# Autodesk Inventor assembly: Shifter
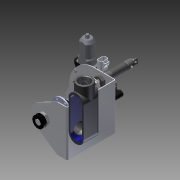
[picture p0: Inventor's stored thumbnail of the model, 180x180]
Saved by Autodesk Inventor 2015 (Build 190159000, 159)
## iProperties
Created: 2015-01-23
Part Number: Shifter
Document SubType Name: Assembly
Designer: Guest
Author: Guest
## Documents named in this file (22)
- C:\Users\Brian\Documents\GitHub\FIRST-Team-1719-CAD-Team\2015 Robot CAD\Devices\Extender\Shifter\Shifter.iam
- C:\Users\Brian\Documents\GitHub\FIRST-Team-1719-CAD-Team\2015 Robot CAD\Devices\Extender\Shifter\ND Motor Left.ipt
- C:\Users\Brian\Documents\GitHub\FIRST-Team-1719-CAD-Team\2015 Robot CAD\Devices\Extender\Shifter\Motor Mount.ipt
- C:\Users\Brian\Documents\GitHub\FIRST-Team-1719-CAD-Team\2015 Robot CAD\Devices\Extender\Shifter\Motor Bolt Nut.ipt
- C:\Users\Brian\Documents\GitHub\FIRST-Team-1719-CAD-Team\2015 Robot CAD\Devices\Extender\Shifter\Motor Bolt.ipt
- C:\Users\Brian\Documents\GitHub\FIRST-Team-1719-CAD-Team\2015 Robot CAD\Devices\Extender\Shifter\Piston\D_9.ipt
- C:\Users\Brian\Documents\GitHub\FIRST-Team-1719-CAD-Team\2015 Robot CAD\Devices\Extender\Shifter\Piston.iam
- C:\Users\Brian\Documents\GitHub\FIRST-Team-1719-CAD-Team\2015 Robot CAD\Devices\Extender\Shifter\Hub.ipt
- C:\Users\Brian\Documents\GitHub\FIRST-Team-1719-CAD-Team\2015 Robot CAD\Devices\Extender\Shifter\Access Fitting.ipt
- C:\Users\Brian\Documents\GitHub\FIRST-Team-1719-CAD-Team\2015 Robot CAD\Devices\Extender\Shifter\Piston Bore Nut.ipt
- C:\Users\Brian\Documents\GitHub\FIRST-Team-1719-CAD-Team\2015 Robot CAD\Devices\Extender\Shifter\Bottom Hub Plate.ipt
- C:\Users\Brian\Documents\GitHub\FIRST-Team-1719-CAD-Team\2015 Robot CAD\Devices\Extender\Shifter\Spacer.ipt
- C:\Users\Brian\Documents\GitHub\FIRST-Team-1719-CAD-Team\2015 Robot CAD\Devices\Extender\Shifter\Upper Hub Plate.ipt
- C:\Users\Brian\Documents\GitHub\FIRST-Team-1719-CAD-Team\2015 Robot CAD\Devices\Extender\Shifter\Flanged Bushing.ipt
- C:\Users\Brian\Documents\GitHub\FIRST-Team-1719-CAD-Team\2015 Robot CAD\Devices\Extender\Shifter\1 4-20 Bolt.ipt
- C:\Users\Brian\Documents\GitHub\FIRST-Team-1719-CAD-Team\2015 Robot CAD\Devices\Extender\Shifter\1 4-20 Nut.ipt
- C:\Users\Brian\Documents\GitHub\FIRST-Team-1719-CAD-Team\2015 Robot CAD\Devices\Extender\Shifter\625 Key Hub.ipt
- C:\Users\Brian\Documents\GitHub\FIRST-Team-1719-CAD-Team\2015 Robot CAD\Devices\Extender\Shifter\5 16 Shaft.ipt
- C:\Users\Brian\Documents\GitHub\FIRST-Team-1719-CAD-Team\2015 Robot CAD\Devices\Extender\Shifter\Shaft Collar.ipt
- C:\Users\Brian\Documents\GitHub\FIRST-Team-1719-CAD-Team\2015 Robot CAD\Devices\Extender\Shifter\Bearing.ipt
- C:\Users\Brian\Documents\GitHub\FIRST-Team-1719-CAD-Team\2015 Robot CAD\Devices\Extender\Shifter\Hub Key.ipt
- C:\Users\Brian\Documents\GitHub\FIRST-Team-1719-CAD-Team\2015 Robot CAD\Devices\Extender\Shifter\Spool Key.ipt
## Components (38 placed, 21 different names)
1. ND Motor Left:1 — Flush:1, Mate:5, Mate:8, Mate:9, Mate:17, Mate:63, Mate:68
2. Motor Mount:1 — Flush:1, Mate:1, Mate:2, Mate:3, Mate:4, Mate:13, Mate:14, Mate:15, Mate:16, Mate:55, Angle:4, Mate:62, Angle:8, Angle:9
3. Motor Bolt Nut:1 — Mate:5, Mate:6
4. Motor Bolt Nut:2 — Mate:7, Mate:8
5. Motor Bolt:1 — Flush:2, Mate:1, Mate:2, Mate:10, Mate:68
6. Motor Bolt:2 — Flush:3, Mate:4, Mate:6
7. Motor Bolt:3 — Flush:2, Flush:3, Mate:3, Mate:7, Mate:63
8. Motor Bolt Nut:3 — Mate:9, Mate:10
9. D_9:1 — Mate:11, Flush:5, Mate:16
10. Piston:1 [sub-assembly] — Flush:4, Mate:11, Mate:13, Mate:14, Angle:1, Mate:20, Mate:24, Flush:9, Angle:5, Mate:67, Flush:17, Mate:69
11. D_9:2 — Mate:12, Flush:5
12. Piston:2 [sub-assembly] — Flush:4, Mate:12, Mate:15, Angle:1, Mate:18, Mate:22, Flush:17
13. Hub:1 — Mate:17, Mate:31, Mate:42, Angle:2, Mate:52, Angle:3
14. Piston Bore Nut:1 — Mate:18
15. Piston Bore Nut:2 — Mate:20, Flush:6, Mate:69
16. Piston Bore Nut:3 — Mate:22, Mate:23
17. Piston Bore Nut:4 — Mate:24, Mate:25, Flush:9
18. Bottom Hub Plate:1 — Flush:6, Mate:23, Mate:25, Flush:7, Mate:36, Mate:64, Mate:65, Mate:67
19. Spacer:1 — Flush:7, Flush:8, Mate:27, Mate:28, Mate:64, Mate:65
20. Upper Hub Plate:1 — Flush:8, Mate:27, Mate:28, Mate:29, Mate:30, Mate:31, Mate:32, Mate:33, Mate:34, Mate:35, Mate:39
21. Flanged Bushing:1 — Mate:29, Mate:30, Mate:54, Mate:66
22. 1 4-20 Bolt:1 — Flush:12, Mate:34, Mate:38
23. 1 4-20 Bolt:2 — Flush:10, Mate:33, Mate:41
24. 1 4-20 Bolt:3 — Flush:11, Flush:12, Mate:35, Mate:37
25. 1 4-20 Bolt:4 — Flush:10, Flush:11, Mate:32, Mate:36, Mate:40
26. 1 4-20 Nut:1 — Flush:13, Flush:14, Mate:39, Mate:40
27. 1 4-20 Nut:2 — Flush:14, Flush:15, Mate:38
28. 1 4-20 Nut:3 — Flush:15, Mate:37
29. 1 4-20 Nut:4 — Flush:13, Mate:41
30. 625 Key Hub:1 — Mate:42, Mate:43, Mate:44, Flush:16, Mate:45, Mate:46, Mate:56
31. 625 Key Hub:2 — Mate:43, Mate:44, Flush:16, Angle:2, Mate:48, Mate:49, Mate:50
32. 5 16 Shaft:1 — Mate:52, Angle:3, Mate:57, Angle:6, Angle:7, Mate:66, Flush:19, Angle:9, Mate:70, Mate:71
33. Shaft Collar:1 — Mate:45, Mate:46, Mate:54, Angle:7, Mate:73
34. Shaft Collar:2 — Mate:48, Mate:51, Angle:6, Flush:19, Mate:58
35. Bearing:1 — Mate:49, Mate:50, Mate:51, Mate:62, Mate:72
36. Access Fitting:1 — Mate:55, Mate:56, Mate:61, Angle:8
37. Hub Key:1 — Flush:20, Flush:21, Mate:71, Mate:73
38. Spool Key:1 — Flush:20, Flush:21, Mate:70, Mate:72
## Relationships (97: Mate 68, Flush 20, Angle 9)
- Flush:1: ND Motor Left:1 ↔ Motor Mount:1
- Flush:2: Motor Bolt:1 ↔ Motor Bolt:3
- Flush:3: Motor Bolt:2 ↔ Motor Bolt:3
- Mate:1: Motor Mount:1 ↔ Motor Bolt:1
- Mate:2: Motor Mount:1 ↔ Motor Bolt:1
- Mate:3: Motor Mount:1 ↔ Motor Bolt:3
- Mate:4: Motor Mount:1 ↔ Motor Bolt:2
- Mate:5: ND Motor Left:1 ↔ Motor Bolt Nut:1
- Mate:6: Motor Bolt Nut:1 ↔ Motor Bolt:2
- Mate:7: Motor Bolt Nut:2 ↔ Motor Bolt:3
- Mate:8: ND Motor Left:1 ↔ Motor Bolt Nut:2
- Mate:9: ND Motor Left:1 ↔ Motor Bolt Nut:3
- Mate:10: Motor Bolt:1 ↔ Motor Bolt Nut:3
- Flush:4: Piston:1 ↔ Piston:2
- Mate:11: D_9:1 ↔ Piston:1
- Mate:12: D_9:2 ↔ Piston:2
- Mate:13: Motor Mount:1 ↔ Piston:1
- Mate:14: Motor Mount:1 ↔ Piston:1
- Mate:15: Motor Mount:1 ↔ Piston:2
- Flush:5: D_9:1 ↔ D_9:2
- Mate:16: Motor Mount:1 ↔ D_9:1
- Angle:1 (0 deg): Piston:1 ↔ Piston:2
- Mate:17: ND Motor Left:1 ↔ Hub:1
- Mate:18: Piston:2 ↔ Piston Bore Nut:1
- Mate:20: Piston:1 ↔ Piston Bore Nut:2
- Flush:6: Piston Bore Nut:2 ↔ Bottom Hub Plate:1
- Mate:22: Piston:2 ↔ Piston Bore Nut:3
- Mate:23: Piston Bore Nut:3 ↔ Bottom Hub Plate:1
- Mate:24: Piston:1 ↔ Piston Bore Nut:4
- Mate:25: Piston Bore Nut:4 ↔ Bottom Hub Plate:1
- Flush:7: Bottom Hub Plate:1 ↔ Spacer:1
- Flush:8: Spacer:1 ↔ Upper Hub Plate:1
- Mate:27: Spacer:1 ↔ Upper Hub Plate:1
- Mate:28: Spacer:1 ↔ Upper Hub Plate:1
- Flush:9 (-2.4892 mm): Piston:1 ↔ Piston Bore Nut:4
- Mate:29: Upper Hub Plate:1 ↔ Flanged Bushing:1
- Mate:30: Upper Hub Plate:1 ↔ Flanged Bushing:1
- Mate:31 (6.35 mm): Hub:1 ↔ Upper Hub Plate:1
- Flush:10: 1 4-20 Bolt:2 ↔ 1 4-20 Bolt:4
- Flush:11: 1 4-20 Bolt:3 ↔ 1 4-20 Bolt:4
- Flush:12: 1 4-20 Bolt:1 ↔ 1 4-20 Bolt:3
- Mate:32: Upper Hub Plate:1 ↔ 1 4-20 Bolt:4
- Mate:33: Upper Hub Plate:1 ↔ 1 4-20 Bolt:2
- Mate:34: Upper Hub Plate:1 ↔ 1 4-20 Bolt:1
- Mate:35: Upper Hub Plate:1 ↔ 1 4-20 Bolt:3
- Mate:36: Bottom Hub Plate:1 ↔ 1 4-20 Bolt:4
- Flush:13: 1 4-20 Nut:1 ↔ 1 4-20 Nut:4
- Flush:14: 1 4-20 Nut:1 ↔ 1 4-20 Nut:2
- Flush:15: 1 4-20 Nut:2 ↔ 1 4-20 Nut:3
- Mate:37: 1 4-20 Bolt:3 ↔ 1 4-20 Nut:3
- Mate:38: 1 4-20 Bolt:1 ↔ 1 4-20 Nut:2
- Mate:39: Upper Hub Plate:1 ↔ 1 4-20 Nut:1
- Mate:40: 1 4-20 Bolt:4 ↔ 1 4-20 Nut:1
- Mate:41: 1 4-20 Bolt:2 ↔ 1 4-20 Nut:4
- Mate:42: Hub:1 ↔ 625 Key Hub:1
- Mate:43: 625 Key Hub:1 ↔ 625 Key Hub:2
- Mate:44: 625 Key Hub:1 ↔ 625 Key Hub:2
- Flush:16: 625 Key Hub:1 ↔ 625 Key Hub:2
- Angle:2 (0 deg): Hub:1 ↔ 625 Key Hub:2
- Mate:45: 625 Key Hub:1 ↔ Shaft Collar:1
- Mate:46: 625 Key Hub:1 ↔ Shaft Collar:1
- Mate:48: 625 Key Hub:2 ↔ Shaft Collar:2
- Mate:49: 625 Key Hub:2 ↔ Bearing:1
- Mate:50: 625 Key Hub:2 ↔ Bearing:1
- Mate:51: Shaft Collar:2 ↔ Bearing:1
- Mate:52: Hub:1 ↔ 5 16 Shaft:1
- Angle:3 (0 deg): Hub:1 ↔ 5 16 Shaft:1
- Mate:54 (25.4 mm): Flanged Bushing:1 ↔ Shaft Collar:1
- Mate:55: Motor Mount:1 ↔ Access Fitting:1
- Mate:56 (-25.4 mm): 625 Key Hub:1 ↔ Access Fitting:1
- Mate:57: 5 16 Shaft:1
- Mate:58: Shaft Collar:2
- Mate:59
- Mate:60
- Angle:4 (0 deg): Motor Mount:1
- Mate:61: Access Fitting:1
- Mate:62: Motor Mount:1 ↔ Bearing:1
- Mate:63: ND Motor Left:1 ↔ Motor Bolt:3
- Angle:5 (0 deg): Piston:1
- Angle:6 (0 deg): 5 16 Shaft:1 ↔ Shaft Collar:2
- Angle:7 (0 deg): 5 16 Shaft:1 ↔ Shaft Collar:1
- Mate:64: Bottom Hub Plate:1 ↔ Spacer:1
- Mate:65: Bottom Hub Plate:1 ↔ Spacer:1
- Mate:66: Flanged Bushing:1 ↔ 5 16 Shaft:1
- Mate:67: Piston:1 ↔ Bottom Hub Plate:1
- Mate:68: ND Motor Left:1 ↔ Motor Bolt:1
- Flush:17: Piston:1 ↔ Piston:2
- Flush:19: 5 16 Shaft:1 ↔ Shaft Collar:2
- Angle:8 (0 deg): Motor Mount:1 ↔ Access Fitting:1
- Mate:69: Piston:1 ↔ Piston Bore Nut:2
- Angle:9 (0 deg): Motor Mount:1 ↔ 5 16 Shaft:1
- Flush:20: Hub Key:1 ↔ Spool Key:1
- Flush:21: Hub Key:1 ↔ Spool Key:1
- Mate:70: 5 16 Shaft:1 ↔ Spool Key:1
- Mate:71: 5 16 Shaft:1 ↔ Hub Key:1
- Mate:72: Bearing:1 ↔ Spool Key:1
- Mate:73: Shaft Collar:1 ↔ Hub Key:1
